# Autodesk Inventor assembly: Ducky caro
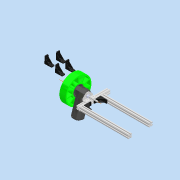
[picture p0: Inventor's stored thumbnail of the model, 180x180]
Saved by Autodesk Inventor 2022 (Build 260153000, 153)
## iProperties
Created: 2022-01-09
Part Number: Ducky caro
Document SubType Name: Assembly
Designer: saji_
Author: saji_
## Documents named in this file (9)
- E:\saji_john\Documents\GitHub\ComputerAidedDesign\2021-22\FTC\#12456 Big Red\Duck carosel\Ducky caro.iam
- E:\saji_john\Documents\GitHub\ComputerAidedDesign\2021-22\FTC\Parts\Custom Parts\15mm Extrusion - 120mm - 90° Ends - 2 Pack.ipt
- E:\saji_john\Documents\GitHub\ComputerAidedDesign\2021-22\FTC\Parts\REV Parts\15mm Extrusion - 120mm - 90° Ends - 2 Pack.ipt
- E:\saji_john\Documents\GitHub\ComputerAidedDesign\2021-22\FTC\#13822 Robovikes\Duck Carousel\REV-41-1300.ipt
- E:\saji_john\Documents\GitHub\ComputerAidedDesign\2021-22\FTC\#13822 Robovikes\Duck Carousel\REV-41-1320.ipt
- E:\saji_john\Documents\GitHub\ComputerAidedDesign\2021-22\FTC\#13822 Robovikes\Duck Carousel\REV-41-1349.ipt
- E:\saji_john\Documents\GitHub\ComputerAidedDesign\2021-22\FTC\#13822 Robovikes\Duck Carousel\REV-41-1433.ipt
- E:\saji_john\Documents\GitHub\ComputerAidedDesign\2021-22\FTC\#13822 Robovikes\Duck Carousel\am-4538 4IN 5mm Hex Compliant Wheel.ipt
- E:\saji_john\Documents\GitHub\ComputerAidedDesign\2021-22\FTC\#13822 Robovikes\Duck Carousel\Slim Shaft Collar - 10 Pack.ipt
## Components (15 placed, 7 different names)
1. 15mm Extrusion - 120mm - 90° Ends - 2 Pack:2 — Mate:3, Mate:4, Mate:5
2. 15mm Extrusion - 120mm - 90° Ends - 2 Pack:3 — Mate:1, Mate:2, Mate:3, Mate:6, Mate:8, Mate:9, Mate:10, Mate:11
3. REV-41-1300:1 — Mate:12, Mate:13, Mate:14, Mate:15, Mate:18
4. REV-41-1320:1 — Mate:5, Mate:6
5. REV-41-1349:1 — Mate:14, Mate:15, Mate:16, Mate:17, Mate:19, Mate:21
6. REV-41-1433:1 — Mate:9, Mate:10, Mate:11, Mate:12, Mate:13, Mate:22
7. REV-41-1320:2 — Mate:7, Mate:8
8. REV-41-1320:3
9. REV-41-1320:4
10. REV-41-1320:5
11. REV-41-1320:6
12. am-4538 4IN 5mm Hex Compliant Wheel:1 — Mate:16, Mate:17, Mate:18, Mate:20
13. Slim Shaft Collar - 10 Pack:1 — Mate:21, Mate:22
14. Slim Shaft Collar - 10 Pack:2 — Mate:19, Mate:20
15. 15mm Extrusion - 120mm - 90° Ends - 2 Pack:1 — Mate:1, Mate:2, Mate:4, Mate:7
## Relationships (22: Mate 22)
- Mate:1: 15mm Extrusion - 120mm - 90° Ends - 2 Pack:3 ↔ 15mm Extrusion - 120mm - 90° Ends - 2 Pack:1
- Mate:2: 15mm Extrusion - 120mm - 90° Ends - 2 Pack:3 ↔ 15mm Extrusion - 120mm - 90° Ends - 2 Pack:1
- Mate:3: 15mm Extrusion - 120mm - 90° Ends - 2 Pack:2 ↔ 15mm Extrusion - 120mm - 90° Ends - 2 Pack:3
- Mate:4 (66.04 mm): 15mm Extrusion - 120mm - 90° Ends - 2 Pack:2 ↔ 15mm Extrusion - 120mm - 90° Ends - 2 Pack:1
- Mate:5: 15mm Extrusion - 120mm - 90° Ends - 2 Pack:2 ↔ REV-41-1320:1
- Mate:6: 15mm Extrusion - 120mm - 90° Ends - 2 Pack:3 ↔ REV-41-1320:1
- Mate:7: REV-41-1320:2 ↔ 15mm Extrusion - 120mm - 90° Ends - 2 Pack:1
- Mate:8: 15mm Extrusion - 120mm - 90° Ends - 2 Pack:3 ↔ REV-41-1320:2
- Mate:9 (25.4 mm): 15mm Extrusion - 120mm - 90° Ends - 2 Pack:3 ↔ REV-41-1433:1
- Mate:10: 15mm Extrusion - 120mm - 90° Ends - 2 Pack:3 ↔ REV-41-1433:1
- Mate:11: 15mm Extrusion - 120mm - 90° Ends - 2 Pack:3 ↔ REV-41-1433:1
- Mate:12: REV-41-1300:1 ↔ REV-41-1433:1
- Mate:13: REV-41-1300:1 ↔ REV-41-1433:1
- Mate:14: REV-41-1300:1 ↔ REV-41-1349:1
- Mate:15: REV-41-1300:1 ↔ REV-41-1349:1
- Mate:16: REV-41-1349:1 ↔ am-4538 4IN 5mm Hex Compliant Wheel:1
- Mate:17: REV-41-1349:1 ↔ am-4538 4IN 5mm Hex Compliant Wheel:1
- Mate:18: REV-41-1300:1 ↔ am-4538 4IN 5mm Hex Compliant Wheel:1
- Mate:19: REV-41-1349:1 ↔ Slim Shaft Collar - 10 Pack:2
- Mate:20: am-4538 4IN 5mm Hex Compliant Wheel:1 ↔ Slim Shaft Collar - 10 Pack:2
- Mate:21: REV-41-1349:1 ↔ Slim Shaft Collar - 10 Pack:1
- Mate:22: REV-41-1433:1 ↔ Slim Shaft Collar - 10 Pack:1
